# Autodesk Inventor assembly: Fixture Assembly
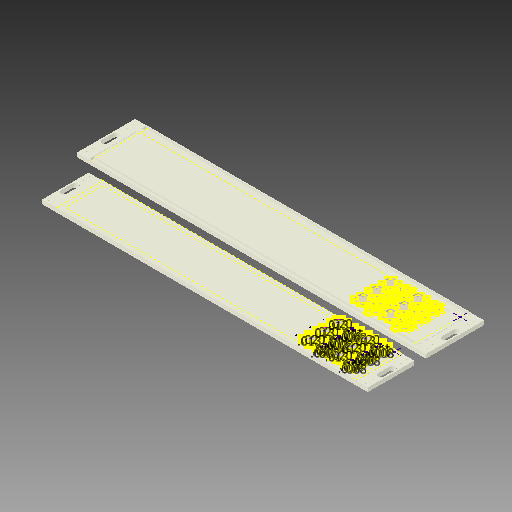
[picture p0: Inventor's stored thumbnail of the model, 512x512]
Saved by Autodesk Inventor 2018 (Build 220112000, 112)
## iProperties
Created: 2016-04-08
Part Number: Fixture Assembly
Document SubType Name: Assembly
Designer: Sam Clay
Author: Sam Clay
## Documents named in this file (6)
- Z:\enclosure\inventor\Fixture Assembly.iam
- Z:\enclosure\inventor\Fixture Base.ipt
- Z:\enclosure\inventor\Case Top Contour Fixture.ipt
- Z:\enclosure\inventor\Case Bottom Contour Fixture.ipt
- Z:\enclosure\inventor\Case Top Pocket Fixture.ipt
- Z:\enclosure\inventor\Case Bottom Pocket Fixture.ipt
## Components (25 placed, 5 different names)
1. Fixture Base:1 — Mate:27, Mate:28, Mate:35, Mate:36, Mate:38, Mate:40
2. Case Top Pocket Fixture:1 — Mate:34, Mate:35, Mate:36, Mate:39
3. Case Bottom Pocket Fixture:1 — Mate:34, Mate:38, Mate:39
4. Case Top Pocket Fixture:3
5. Case Bottom Pocket Fixture:2
6. Case Top Pocket Fixture:4
7. Case Bottom Pocket Fixture:3
8. Case Top Pocket Fixture:5
9. Case Bottom Pocket Fixture:4
10. Case Top Pocket Fixture:6
11. Case Bottom Pocket Fixture:5
12. Case Top Pocket Fixture:7
13. Case Bottom Pocket Fixture:6
14. Case Top Contour Fixture:1 — Mate:27, Mate:28, Mate:31, Mate:32, Mate:40
15. Case Bottom Contour Fixture:16 — Mate:31, Mate:32
16. Case Top Contour Fixture:2
17. Case Bottom Contour Fixture:17
18. Case Top Contour Fixture:3
19. Case Bottom Contour Fixture:18
20. Case Top Contour Fixture:4
21. Case Bottom Contour Fixture:19
22. Case Top Contour Fixture:5
23. Case Bottom Contour Fixture:20
24. Case Top Contour Fixture:6
25. Case Bottom Contour Fixture:21
## Component patterns: (1 elements), (1 elements), (6 elements, first: Case Top Pocket Fixture:1 + Case Bottom Pocket Fixture:1), (6 elements, first: Case Top Contour Fixture:1 + Case Bottom Contour Fixture:16)
## Relationships (10: Mate 10)
- Mate:27 (22.225 mm): Fixture Base:1 ↔ Case Top Contour Fixture:1
- Mate:28 (35.56 mm): Fixture Base:1 ↔ Case Top Contour Fixture:1
- Mate:31: Case Top Contour Fixture:1 ↔ Case Bottom Contour Fixture:16
- Mate:32 (7.8994 mm): Case Top Contour Fixture:1 ↔ Case Bottom Contour Fixture:16
- Mate:34: Case Top Pocket Fixture:1 ↔ Case Bottom Pocket Fixture:1
- Mate:35 (19.05 mm): Fixture Base:1 ↔ Case Top Pocket Fixture:1
- Mate:36 (3.175 mm): Fixture Base:1 ↔ Case Top Pocket Fixture:1
- Mate:38: Fixture Base:1 ↔ Case Bottom Pocket Fixture:1
- Mate:39 (7.8994 mm): Case Top Pocket Fixture:1 ↔ Case Bottom Pocket Fixture:1
- Mate:40 (15.24 mm): Fixture Base:1 ↔ Case Top Contour Fixture:1
